# Autodesk Inventor assembly: HFROLL5
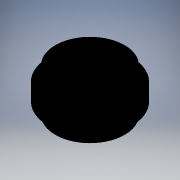
[picture p0: Inventor's stored thumbnail of the model, 180x180]
Saved by Autodesk Inventor 2017.3 (Build 213256000, 256)
## iProperties
Category: PARTsolutions
Company: MISUMI
Part Number: HFROLL5
Catalog Web Link: www.cadenas.de
Description: HFROLL, HFROLLM-Rollers for Aluminum Frames
Vendor: MISUMI
Document SubType Name: Assembly
Designer: partserver
Manufacturer: MISUMI
Mass: 7.74283 g
Surface Area: 39.3032 cm^2
Volume: 7.74283 cm^3
Density: 1 g/cm^3
Title: HFROLL5
Author: Cadenas PARTsolutions
Comments: Rollers for Aluminum Frames
PSOL_IDENT_0: {$CADENAS_DATA\23d-libs\misumi\metric\39_accessories_for_al_extrusions\hfroll_asmtab.prj},182 {VTYP=
PSOL_IDENT_1: 3D},{STYP=ASSTAB},{NB=HFROLL5},{LINA=HFROLL5},{NN=HFROLL, HFROLLM},{DATE=09.09.2019 15:28:13},{GEOMD
PSOL_IDENT_2: ATE=02.06.2016 02:55:28},{VERSION=},{LINEID=10},{WBVAR=MATAC},{WBNUMERIC=}  {NB=HFROLL5},{LINA=HFROL
PSOL_IDENT_3: L5},{KT=DUMMY},{PN=HFROLL5},{MATAC=HFROLL},{STAC=-},{MATR=Nylon 6},{TYPE=HFROLL},{NO=5},{CFSW=6},{AF
PSOL_IDENT_4: S=HFS5},{H=6.0},{D=24},{T=15.0},{TT1=4},{TT2=5},{DD1=29.0},{DD2=9.2},{COLOR=Black},{BEARING=None},{A
PSOL_IDENT_5: CL=16.5},{ACTT3=1.5},{ACD2=9},{ACDD4=6.2},{ACDD5=13},{QAC=1},{PPATH=hfroll/hfroll_templ.prj}
NB: HFROLL5
NN: HFROLL, HFROLLM
NT: Rollers for Aluminum Frames
NBSYN: $PN.
LINA: HFROLL5
CATALOG: Misumi
PN: HFROLL5
MATAC: Nylon 6
STAC: -
MATR: Nylon 6
NO: 5
AFS: HFS5
H: 6
D: 24
T: 15
TT1: 4
TT2: 5
DD1: 29
DD2: 9.2
COLOR: Black
BEARING: Not Provided
ACL: 16.5
ACTT3: 1.5
ACD2: 9
ACDD4: 6.2
ACDD5: 13
QAC: 1
SUPPLIER: MISUMI
ARTICLENO: HFROLL5
BOMINFO: HFROLL5
CREATOR: CADENAS GmbH
## Documents named in this file (3)
- e:\temp\worker_10\temp\exporttempdir_3608_238_MYe2s\format_0\HFROLL5.iam
- e:\temp\worker_10\temp\exporttempdir_3608_238_MYe2s\format_0\HFROLL5_b.ipt
- e:\temp\worker_10\temp\exporttempdir_3608_238_MYe2s\format_0\HFROLL5_a.ipt
## Components (2 placed, 2 different names)
1. HFROLL5_b:1 — 1_XY@1 <-> to_roller_XY@2, 1_Z@1 <-> to_roller_Z@2, 1_YZ@1 <-> to_roller_YZ@2
2. HFROLL5_a:1 — 1_XY@1 <-> to_roller_XY@2, 1_Z@1 <-> to_roller_Z@2, 1_YZ@1 <-> to_roller_YZ@2
## Relationships (3: Mate 2, Angle 1)
- 1_XY@1 <-> to_roller_XY@2 [Mate]: HFROLL5_b:1 ↔ HFROLL5_a:1
- 1_Z@1 <-> to_roller_Z@2 [Mate]: HFROLL5_b:1 ↔ HFROLL5_a:1
- 1_YZ@1 <-> to_roller_YZ@2 [Angle] (0 deg): HFROLL5_b:1 ↔ HFROLL5_a:1
